# Autodesk Inventor assembly: roller
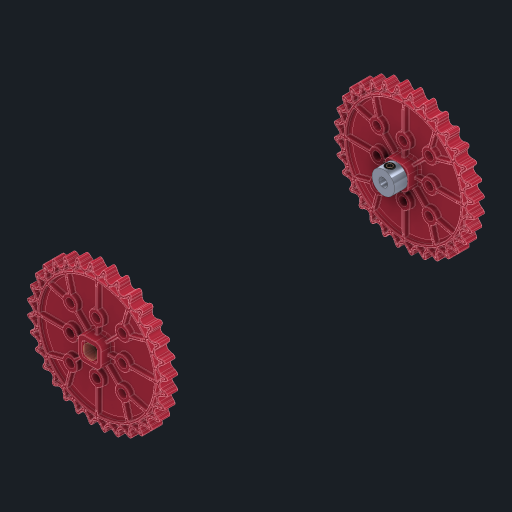
[picture p0: Inventor's stored thumbnail of the model, 512x512]
Saved by Autodesk Inventor 2024 (Build 280153000, 153)
## iProperties
Created: 2023-08-21
Part Number: roller
Document SubType Name: Assembly
Designer: Averey
Author: Averey
## Documents named in this file (4)
- C:\Users\Averey\Documents\vex\cad\scrap_v0.1\intake\roller.iam
- C:\Users\Averey\Documents\vex\cad\VEX-CAD-Inventor-1.41\Motion\Shaft LS\Shaft Collar ipts\Shaft Collar Set Screw.ipt
- C:\Users\Averey\Documents\vex\cad\VEX-CAD-Inventor-1.41\Motion\Sprockets\6P Sprocket.iam
- C:\Users\Averey\Documents\vex\cad\VEX-CAD-Inventor-1.41\Motion\Sprockets\6P Sprocket\6P 32T Sprocket, No Insert.iam
## Components (4 placed, 2 different names)
1. Shaft Collar Set Screw:1 — Insert:6
2. Shaft Collar Set Screw:2 — Insert:7
3. 6P 32T Sprocket, No Insert:3 [sub-assembly] — Insert:6
4. 6P 32T Sprocket, No Insert:4 [sub-assembly] — Insert:7
## Relationships (2: Insert 2)
- Insert:6: Shaft Collar Set Screw:1 ↔ 6P 32T Sprocket, No Insert:3
- Insert:7: Shaft Collar Set Screw:2 ↔ 6P 32T Sprocket, No Insert:4
